# Autodesk Inventor assembly: P80 Mount Assembly V2
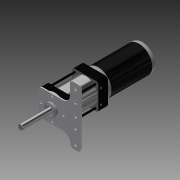
[picture p0: Inventor's stored thumbnail of the model, 180x180]
Saved by Autodesk Inventor 2013 (Build 170138000, 138)
## iProperties
Created: 2013-02-03
Part Number: P80 Mount Assembly V2
Document SubType Name: Assembly
Designer: Arpan
Mass: 3046.27 g
Surface Area: 1230.05 cm^2
Volume: 600.336 cm^3
Density: 5.07428 g/cm^3
Author: Arpan
## Documents named in this file (6)
- C:\Users\Moses\Documents\GitHub\frc2013CAD\Cimber actual\P80 Mount Assembly V2.iam
- C:\Users\Moses\Documents\GitHub\frc2013CAD\Cimber actual\p80 mount plate.ipt
- C:\Users\Moses\Documents\GitHub\frc2013CAD\Cimber actual\1.5 inch bearing.ipt
- C:\Users\Moses\Documents\GitHub\frc2013CAD\Cimber actual\P80 Gearbox\P80 Gearbox 3-stage.iam
- C:\Users\Moses\Documents\GitHub\frc2013CAD\Cimber actual\P80 Gearbox\CIM motor.ipt
- C:\Users\Moses\Documents\GitHub\frc2013CAD\Cimber actual\P80 Spacer.ipt
## Components (5 placed, 5 different names)
1. p80 mount plate:1 — Mate:1, Mate:2, Mate:3, Mate:5, Mate:6, Mate:7
2. 1.5 inch bearing:1 — Mate:1, Mate:2, Insert:1
3. P80 Gearbox 3-stage:1 [sub-assembly] — Insert:1, Mate:3, Mate:4, Insert:2
4. CIM motor:1 — Mate:4, Insert:2
5. P80 Spacer:1 — Mate:5, Mate:6, Mate:7
## Relationships (9: Mate 7, Insert 2)
- Mate:1: p80 mount plate:1 ↔ 1.5 inch bearing:1
- Mate:2: p80 mount plate:1 ↔ 1.5 inch bearing:1
- Insert:1: 1.5 inch bearing:1 ↔ P80 Gearbox 3-stage:1
- Mate:3: p80 mount plate:1 ↔ P80 Gearbox 3-stage:1
- Mate:4: P80 Gearbox 3-stage:1 ↔ CIM motor:1
- Insert:2: P80 Gearbox 3-stage:1 ↔ CIM motor:1
- Mate:5: p80 mount plate:1 ↔ P80 Spacer:1
- Mate:6: p80 mount plate:1 ↔ P80 Spacer:1
- Mate:7: p80 mount plate:1 ↔ P80 Spacer:1
